# Autodesk Inventor assembly: BrushlessMotor_N5065
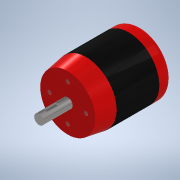
[picture p0: Inventor's stored thumbnail of the model, 180x180]
Saved by Autodesk Inventor 2022.3 (Build 263350000, 350)
## iProperties
Created: 2020-08-28
Part Number: BrushlessMotor_N5065
Document SubType Name: Assembly
Designer: Hagihara Yuya
Mass: 450 g
Surface Area: 188.767 cm^2
Volume: 114.553 cm^3
Author: Hagihara Yuya
## Documents named in this file (3)
- C:\Users\YusukeKunita\Documents\GrabCAD\Development\BasicParts\BrushlessMotor\BrushlessMotor_N5065.iam
- C:\Users\YusukeKunita\Documents\GrabCAD\Development\BasicParts\BrushlessMotor\Stator_N5065.ipt
- C:\Users\YusukeKunita\Documents\GrabCAD\Development\BasicParts\BrushlessMotor\Rotator_N5065.ipt
## Components (2 placed, 2 different names)
1. Stator_N5065:1 — 回転:1
2. Rotator_N5065:1 — 回転:1
## Relationships (1: RevoluteJoint 1)
- 回転:1 [RevoluteJoint]: Stator_N5065:1 ↔ Rotator_N5065:1
